# Autodesk Inventor assembly: Lead Screw Prototype A
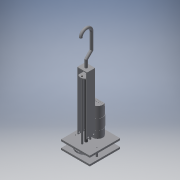
[picture p0: Inventor's stored thumbnail of the model, 180x180]
Saved by Autodesk Inventor 2019 (Build 230136000, 136)
## iProperties
Created: 2018-09-13
Part Number: Lead Screw Prototype A
Document SubType Name: Assembly
Designer: drawing
Author: drawing
## Documents named in this file (18)
- C:\Robotics\CAD\2018-19_CAD\lift assembly\Lead Screw Prototype A.iam
- C:\Robotics\CAD\2018-19_CAD\lift assembly\Part3.ipt
- C:\Robotics\CAD\2018-19_CAD\lift assembly\ActoBotics Bearing .375.ipt
- C:\Robotics\CAD\2018-19_CAD\lift assembly\Tetrix Gear 80T.ipt
- C:\Robotics\CAD\2018-19_CAD\lift assembly\Part2.ipt
- C:\Robotics\CAD\2018-19_CAD\lift assembly\Tetrix Gear 40T.ipt
- C:\Robotics\CAD\2018-19_CAD\lift assembly\Part6.ipt
- C:\Robotics\CAD\2018-19_CAD\lift assembly\Part5.ipt
- C:\Robotics\CAD\2018-19_CAD\lift assembly\Andymark 2964  NeveRest 40 Motor.ipt
- C:\Robotics\CAD\2018-19_CAD\lift assembly\AS 1420 - 1973 - M3 x 6.ipt
- C:\Robotics\CAD\2018-19_CAD\lift assembly\ANSI B18.3 - 6-32 UNC - 0.5(31).ipt
- C:\Robotics\CAD\2018-19_CAD\lift assembly\Part9.ipt
- Z:\Sadler\Austin\95082A641.iam
- C:\Robotics\CAD\2018-19_CAD\lift assembly\Tetrix Hub - axle.ipt
- C:\Robotics\CAD\2018-19_CAD\lift assembly\Tetrix hub - motor.ipt
- C:\Robotics\CAD\2018-19_CAD\lift assembly\Part11.ipt
- C:\Robotics\CAD\2018-19_CAD\lift assembly\ANSI B18.3 - 1_4-20 UNC - 0.75(31).ipt
- C:\Robotics\CAD\2018-19_CAD\lift assembly\Part12.ipt
## Components (29 placed, 17 different names)
1. Part3:1 — Insert:1, Insert:7, Mate:3, Insert:10, Insert:11, Insert:13, Insert:14, Mate:8, Mate:9, Mate:10, Insert:15, Insert:16, Insert:17, Insert:18, Insert:19, Insert:20, Insert:21, Insert:22, Angle:1
2. ActoBotics Bearing .375:1 — Insert:1, Mate:11
3. Part3:2 — Insert:9, Insert:12, Mate:4
4. ActoBotics Bearing .375:2 — Insert:9
5. Tetrix Gear 80T:1 — Mate:1, Flush:1, Insert:26
6. Part2:1 — Insert:7, Mate:1, Mate:4, Mate:12, Insert:31
7. Tetrix Gear 40T:1 — Mate:3, Flush:1, Insert:27
8. Part6:1 — Insert:10
9. Part6:2 — Insert:11, Insert:12
10. Part5:1 — Insert:13, Mate:5, Mate:13
11. Part5:2 — Insert:14, Mate:6
12. 95082A641:1 [sub-assembly] — Mate:5, Mate:6, Insert:28, Flush:2, Mate:12
13. Andymark 2964  NeveRest 40 Motor:1 — Mate:8, Mate:9, Mate:10
14. AS 1420 - Metric M3 x 6:1 — Insert:19
15. AS 1420 - Metric M3 x 6:2 — Insert:17
16. AS 1420 - Metric M3 x 6:3 — Insert:18
17. AS 1420 - Metric M3 x 6:4 — Insert:20
18. AS 1420 - Metric M3 x 6:5 — Insert:15
19. AS 1420 - Metric M3 x 6:6 — Insert:16
20. Hexagon Socket Head Cap Screw - Inch No. 6 - 32 UNC - 1/2:1 — Insert:21
21. Hexagon Socket Head Cap Screw - Inch No. 6 - 32 UNC - 1/2:2 — Insert:22
22. Part9:1 — Angle:1, Insert:29
23. Tetrix Hub - axle:1 — Insert:26, Mate:11
24. Tetrix hub - motor:1 — Insert:27
25. Part11:1 — Insert:28, Flush:2, Insert:29, Insert:30
26. Hexagon Socket Head Cap Screw - Inch 1/4 - 20 UNC - 3/4:1 — Insert:30
27. Part12:1 — Insert:31, Mate:13, Insert:32, Insert:33
28. Hexagon Socket Head Cap Screw - Inch No. 6 - 32 UNC - 1/2:3 — Insert:32
29. Hexagon Socket Head Cap Screw - Inch No. 6 - 32 UNC - 1/2:4 — Insert:33
## Relationships (38: Insert 24, Mate 11, Flush 2, Angle 1)
- Insert:1: Part3:1 ↔ ActoBotics Bearing .375:1
- Insert:7: Part3:1 ↔ Part2:1
- Mate:1: Tetrix Gear 80T:1 ↔ Part2:1
- Insert:9: Part3:2 ↔ ActoBotics Bearing .375:2
- Mate:3: Part3:1 ↔ Tetrix Gear 40T:1
- Flush:1: Tetrix Gear 80T:1 ↔ Tetrix Gear 40T:1
- Insert:10: Part3:1 ↔ Part6:1
- Insert:11: Part3:1 ↔ Part6:2
- Insert:12: Part3:2 ↔ Part6:2
- Mate:4: Part3:2 ↔ Part2:1
- Insert:13: Part3:1 ↔ Part5:1
- Insert:14: Part3:1 ↔ Part5:2
- Mate:5: Part5:1 ↔ 95082A641:1
- Mate:6: Part5:2 ↔ 95082A641:1
- Mate:8: Part3:1 ↔ Andymark 2964  NeveRest 40 Motor:1
- Mate:9: Part3:1 ↔ Andymark 2964  NeveRest 40 Motor:1
- Mate:10: Part3:1 ↔ Andymark 2964  NeveRest 40 Motor:1
- Insert:15: Part3:1 ↔ AS 1420 - Metric M3 x 6:5
- Insert:16: Part3:1 ↔ AS 1420 - Metric M3 x 6:6
- Insert:17: Part3:1 ↔ AS 1420 - Metric M3 x 6:2
- Insert:18: Part3:1 ↔ AS 1420 - Metric M3 x 6:3
- Insert:19: Part3:1 ↔ AS 1420 - Metric M3 x 6:1
- Insert:20: Part3:1 ↔ AS 1420 - Metric M3 x 6:4
- Insert:21: Part3:1 ↔ Hexagon Socket Head Cap Screw - Inch No. 6 - 32 UNC - 1/2:1
- Insert:22: Part3:1 ↔ Hexagon Socket Head Cap Screw - Inch No. 6 - 32 UNC - 1/2:2
- Angle:1 (180 deg): Part3:1 ↔ Part9:1
- Insert:26: Tetrix Gear 80T:1 ↔ Tetrix Hub - axle:1
- Insert:27: Tetrix Gear 40T:1 ↔ Tetrix hub - motor:1
- Mate:11: ActoBotics Bearing .375:1 ↔ Tetrix Hub - axle:1
- Insert:28: 95082A641:1 ↔ Part11:1
- Flush:2: 95082A641:1 ↔ Part11:1
- Insert:29: Part9:1 ↔ Part11:1
- Insert:30: Part11:1 ↔ Hexagon Socket Head Cap Screw - Inch 1/4 - 20 UNC - 3/4:1
- Mate:12: Part2:1 ↔ 95082A641:1
- Insert:31: Part2:1 ↔ Part12:1
- Mate:13: Part5:1 ↔ Part12:1
- Insert:32: Part12:1 ↔ Hexagon Socket Head Cap Screw - Inch No. 6 - 32 UNC - 1/2:3
- Insert:33: Part12:1 ↔ Hexagon Socket Head Cap Screw - Inch No. 6 - 32 UNC - 1/2:4
